# Autodesk Inventor assembly: beep_rgb_ir_assembled_2
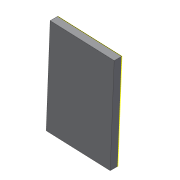
[picture p0: Inventor's stored thumbnail of the model, 180x180]
Saved by Autodesk Inventor 2014 (Build 180170000, 170)
## iProperties
Created: 2013-08-25
Part Number: beep_rgb_ir_assembled_2
Document SubType Name: Assembly
Designer: Felix
Author: Felix
## Documents named in this file (4)
- C:\Users\Felix\Desktop\Beep\Hardware\3D-CAD\parts\electronic\BEEP\beep_rgb_ir_assembled_2.iam
- C:\Users\Felix\Desktop\Beep\Hardware\3D-CAD\parts\electronic\BEEP\beep_rgb_ir.ipt
- C:\Users\Felix\Desktop\Beep\Hardware\3D-CAD\parts\electronic\BEEP\components\HSDL-9100-024\HSDL-9100.iam
- C:\Users\Felix\Desktop\Beep\Hardware\3D-CAD\parts\electronic\BEEP\components\5050 LED\5050_LED.ipt
## Components (3 placed, 3 different names)
1. beep_rgb_ir:1 — Passend:5, Passend:13
2. HSDL-9100:1 [sub-assembly] — Passend:5
3. 5050_LED:1 — Passend:13
## Relationships (2: Mate 2)
- Passend:5 [Mate]: beep_rgb_ir:1 ↔ HSDL-9100:1
- Passend:13 [Mate]: beep_rgb_ir:1 ↔ 5050_LED:1
